# Autodesk Inventor assembly: Picker Tool
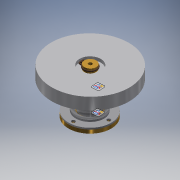
[picture p0: Inventor's stored thumbnail of the model, 180x180]
Saved by Autodesk Inventor 2019.4 (Build 234330000, 330)
## iProperties
Created: 2021-01-08
Part Number: Picker Tool
Document SubType Name: Assembly
Designer: caleb
Author: caleb
## Documents named in this file (5)
- C:\Users\cfang\Desktop\nebraska-silicon-lab\CAD\ETL\Module Assembly\Picker Tool\Picker Tool.iam
- C:\Users\cfang\Desktop\nebraska-silicon-lab\CAD\ETL\Module Assembly\Picker Tool\Picker Base.ipt
- C:\Users\cfang\Desktop\nebraska-silicon-lab\CAD\ETL\Module Assembly\Picker Tool\Picker Spool.ipt
- C:\Users\cfang\Desktop\nebraska-silicon-lab\CAD\ETL\Module Assembly\Picker Tool\Bellows Assembly.iam
- C:\Users\cfang\Desktop\nebraska-silicon-lab\CAD\ETL\Module Assembly\Picker Tool\91590A115_STAINLESS STEEL EXTERNAL RETAINING RING.ipt
## Components (4 placed, 4 different names)
1. Picker Base:1 — Cylindrical:1, Cylindrical:2, Mate:1
2. Picker Spool:1 — Cylindrical:1, Mate:2, Insert:1
3. Bellows Assembly:1 [sub-assembly] — Cylindrical:2, Mate:1, Mate:2
4. 91590A115_STAINLESS STEEL EXTERNAL RETAINING RING:1 — Insert:1
## Relationships (5: CylindricalJoint 2, Mate 2, Insert 1)
- Cylindrical:1: Picker Base:1 ↔ Picker Spool:1
- Cylindrical:2: Picker Base:1 ↔ Bellows Assembly:1
- Mate:1: Picker Base:1 ↔ Bellows Assembly:1
- Mate:2: Picker Spool:1 ↔ Bellows Assembly:1
- Insert:1: Picker Spool:1 ↔ 91590A115_STAINLESS STEEL EXTERNAL RETAINING RING:1
